# Autodesk Inventor assembly: Samenstelling
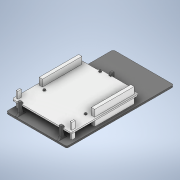
[picture p0: Inventor's stored thumbnail of the model, 180x180]
Saved by Autodesk Inventor 2022 (Build 260153000, 153)
## iProperties
Created: 2022-02-18
Part Number: Samenstelling
Document SubType Name: Assembly
Designer: woutr
Author: woutr
## Documents named in this file (3)
- C:\Users\woutr\OneDrive\Documenten\Inventor\Project Klascomfortmonitoring\Samenstelling.iam
- C:\Users\woutr\OneDrive\Documenten\Inventor\Project Klascomfortmonitoring\Bodemplaat.ipt
- C:\Users\woutr\OneDrive\Documenten\Inventor\Project Klascomfortmonitoring\Microcontroller.ipt
## Components (2 placed, 2 different names)
1. Bodemplaat:1 — Mate:1, Mate:2, Mate:3
2. Microcontroller:1 — Mate:1, Mate:2, Mate:3
## Relationships (3: Mate 3)
- Mate:1: Bodemplaat:1 ↔ Microcontroller:1
- Mate:2: Bodemplaat:1 ↔ Microcontroller:1
- Mate:3: Bodemplaat:1 ↔ Microcontroller:1
